# Autodesk Inventor assembly: Build Platform Assembly 1.0
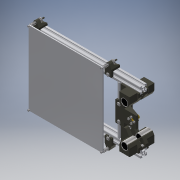
[picture p0: Inventor's stored thumbnail of the model, 180x180]
Saved by Autodesk Inventor 2016 (Build 200138000, 138)
## iProperties
Created: 2017-04-13
Part Number: Build Platform Assembly 1.0
Document SubType Name: Assembly
Designer: Scott
Author: Scott
## Documents named in this file (16)
- E:\Scott Projects\3D Printing\CoreXY\Build Platform Assembly 1.0.iam
- E:\Scott Projects\3D Printing\CoreXY\2020 Extrusion - Bed rear.ipt
- E:\Scott Projects\3D Printing\CoreXY\Z Axis Bearing Holder 1.0.ipt
- E:\Scott Projects\3D Printing\CoreXY\2020 Extrusion - Bed sides.ipt
- E:\Scott Projects\3D Printing\CoreXY\LM12UU.ipt
- E:\Scott Projects\3D Printing\CoreXY\Heated Bed.ipt
- E:\Scott Projects\3D Printing\CoreXY\Mk2 Heat Bed Bracket.ipt
- C:\Users\Scott\Documents\Inventor\Content Center Files\R2016\en-US\ANSI B18.3.4M(1)\ANSI B18.3.4M - M5 x 0.8 x 10(2).ipt
- C:\Users\Scott\Documents\Inventor\Content Center Files\R2016\en-US\ANSI B18.3.1M(1)\ANSI B18.3.1M - M3x0.5 x 40(2).ipt
- E:\Scott Projects\3D Printing\CoreXY\Bed spring.ipt
- E:\Scott Projects\3D Printing\CoreXY\Bed Thumb Screw.ipt
- E:\Scott Projects\3D Printing\CoreXY\Z Nut Braket 1.0.ipt
- E:\Scott Projects\3D Printing\CoreXY\Trapezoidal lead screw Nut tr8x8-4.ipt
- C:\Users\Scott\Documents\Inventor\Content Center Files\R2016\en-US\ANSI B18.3.1M(1)\ANSI B18.3.1M - M3x0.5 x 12(2).ipt
- C:\Users\Scott\Documents\Inventor\Content Center Files\R2016\en-US\ISO 4032(2)\ISO 4032 - M3 - ISO.ipt
- E:\Scott Projects\3D Printing\CoreXY\HyperCube parameters.xlsx
## Components (56 placed, 14 different names)
1. 2020 Extrusion - Bed rear:1 — Flush:1, Flush:2, Flush:3, Mate:1, Flush:4, Mate:2, Mate:3, Mate:4, Flush:5, Mate:10, Mate:28, Mate:29
2. Z Axis Bearing Holder 1.0:1 — Mate:3, Mate:4, Flush:5, Mate:5, Mate:6, Flush:7, Insert:2, Insert:4, Insert:26, Insert:27, Insert:28, Insert:29
3. Z Axis Bearing Holder 1.0:2 — Mate:1, Flush:4, Mate:2, Mate:7, Mate:8, Flush:6, Insert:1, Insert:3, Insert:22, Insert:23, Insert:24, Insert:25
4. 2020 Extrusion - Bed sides:1 — Mate:5, Mate:6, Flush:7, Mate:9, Mate:18, Mate:19, Mate:21, Mate:22
5. 2020 Extrusion - Bed sides:2 — Mate:7, Mate:8, Flush:6, Mate:12, Mate:13, Mate:15, Mate:16
6. LM12UU:1 — Insert:4
7. LM12UU:2 — Insert:3
8. LM12UU:3 — Insert:2
9. LM12UU:4 — Insert:1, Mate:11
10. Heated Bed:1 — Mate:9, Mate:10, Mate:11, Mate:14, Mate:17, Mate:20, Mate:23, Insert:13, Insert:14, Insert:15, Insert:16
11. Mk2 Heat Bed Bracket:1 — Mate:12, Mate:13, Mate:14, Insert:11, Insert:12, Flush:9, Insert:20
12. Mk2 Heat Bed Bracket:2 — Mate:15, Mate:16, Mate:17, Insert:9, Insert:10, Flush:8, Insert:19
13. Mk2 Heat Bed Bracket:3 — Mate:21, Mate:22, Mate:23, Insert:5, Flush:10, Insert:18, Insert:21
14. Mk2 Heat Bed Bracket:4 — Mate:18, Mate:19, Mate:20, Insert:7, Insert:8, Flush:11, Insert:17
15. Broached Hexagon Socket Button Head Cap Screw - Metric M5 x 0.8 x 10:1 — Insert:9
16. Broached Hexagon Socket Button Head Cap Screw - Metric M5 x 0.8 x 10:2 — Insert:12
17. Broached Hexagon Socket Button Head Cap Screw - Metric M5 x 0.8 x 10:3 — Insert:8
18. Broached Hexagon Socket Button Head Cap Screw - Metric M5 x 0.8 x 10:4 — Insert:11
19. Broached Hexagon Socket Button Head Cap Screw - Metric M5 x 0.8 x 10:5 — Insert:7
20. Broached Hexagon Socket Button Head Cap Screw - Metric M5 x 0.8 x 10:6 — Insert:10
21. Broached Hexagon Socket Button Head Cap Screw - Metric M5 x 0.8 x 10:7 — Insert:5
22. Broached Hexagon Socket Button Head Cap Screw - Metric M5 x 0.8 x 10:8 — Insert:21
23. Broached Socket Head Cap Screw - Metric M3x0.5 x 40:1 — Insert:16, Mate:27
24. Broached Socket Head Cap Screw - Metric M3x0.5 x 40:2 — Insert:15, Mate:26
25. Broached Socket Head Cap Screw - Metric M3x0.5 x 40:3 — Insert:14, Mate:25
26. Broached Socket Head Cap Screw - Metric M3x0.5 x 40:4 — Insert:13, Mate:24
27. Bed spring:1 — Mate:24, Flush:8
28. Bed spring:2 — Mate:25, Flush:9
29. Bed spring:3 — Mate:26, Flush:10
30. Bed spring:4 — Mate:27, Flush:11
31. Bed Thumb Screw:1 — Insert:19
32. Bed Thumb Screw:2 — Insert:17
33. Bed Thumb Screw:3 — Insert:20
34. Bed Thumb Screw:4 — Insert:18
35. Broached Hexagon Socket Button Head Cap Screw - Metric M5 x 0.8 x 10:9 — Insert:22
36. Broached Hexagon Socket Button Head Cap Screw - Metric M5 x 0.8 x 10:10 — Insert:23
37. Broached Hexagon Socket Button Head Cap Screw - Metric M5 x 0.8 x 10:11 — Insert:24
38. Broached Hexagon Socket Button Head Cap Screw - Metric M5 x 0.8 x 10:12 — Insert:25
39. Broached Hexagon Socket Button Head Cap Screw - Metric M5 x 0.8 x 10:13 — Insert:29
40. Broached Hexagon Socket Button Head Cap Screw - Metric M5 x 0.8 x 10:14 — Insert:28
41. Broached Hexagon Socket Button Head Cap Screw - Metric M5 x 0.8 x 10:15 — Insert:27
42. Broached Hexagon Socket Button Head Cap Screw - Metric M5 x 0.8 x 10:16 — Insert:26
43. Z Nut Braket 1.0:1 — Mate:28, Mate:29, Flush:12, Insert:30, Insert:31, Insert:32, Insert:33, Mate:31, Mate:34, Mate:35, Mate:37, Mate:39, Angle:1, Angle:2, Angle:3, Angle:4, Mate:41
44. Broached Hexagon Socket Button Head Cap Screw - Metric M5 x 0.8 x 10:17 — Insert:31
45. Broached Hexagon Socket Button Head Cap Screw - Metric M5 x 0.8 x 10:18 — Insert:30
46. Broached Hexagon Socket Button Head Cap Screw - Metric M5 x 0.8 x 10:19 — Insert:32
47. Broached Hexagon Socket Button Head Cap Screw - Metric M5 x 0.8 x 10:20 — Insert:33
48. Trapezoidal lead screw Nut tr8x8-4:1 — Mate:30, Mate:31, Mate:32, Mate:33, Mate:36, Mate:38, Mate:40, Insert:34, Insert:35, Insert:36, Insert:37, Mate:41
49. Broached Socket Head Cap Screw - Metric M3x0.5 x 12:1 — Mate:33, Mate:34
50. Broached Socket Head Cap Screw - Metric M3x0.5 x 12:2 — Mate:39, Mate:40
51. Broached Socket Head Cap Screw - Metric M3x0.5 x 12:3 — Mate:37, Mate:38
52. Broached Socket Head Cap Screw - Metric M3x0.5 x 12:4 — Mate:35, Mate:36
53. ISO 4032 M3:1 — Insert:34, Angle:1
54. ISO 4032 M3:2 — Insert:36, Angle:4
55. ISO 4032 M3:3 — Insert:37, Angle:2
56. ISO 4032 M3:4 — Insert:35, Angle:3
## Relationships (93: Mate 41, Insert 36, Flush 12, Angle 4)
- Flush:1: 2020 Extrusion - Bed rear:1
- Flush:2 (0.2 mm): 2020 Extrusion - Bed rear:1
- Flush:3: 2020 Extrusion - Bed rear:1
- Mate:1: 2020 Extrusion - Bed rear:1 ↔ Z Axis Bearing Holder 1.0:2
- Flush:4: 2020 Extrusion - Bed rear:1 ↔ Z Axis Bearing Holder 1.0:2
- Mate:2 (0.2 mm): 2020 Extrusion - Bed rear:1 ↔ Z Axis Bearing Holder 1.0:2
- Mate:3: 2020 Extrusion - Bed rear:1 ↔ Z Axis Bearing Holder 1.0:1
- Mate:4: 2020 Extrusion - Bed rear:1 ↔ Z Axis Bearing Holder 1.0:1
- Flush:5: 2020 Extrusion - Bed rear:1 ↔ Z Axis Bearing Holder 1.0:1
- Mate:5: Z Axis Bearing Holder 1.0:1 ↔ 2020 Extrusion - Bed sides:1
- Mate:6 (0.2 mm): Z Axis Bearing Holder 1.0:1 ↔ 2020 Extrusion - Bed sides:1
- Mate:7: Z Axis Bearing Holder 1.0:2 ↔ 2020 Extrusion - Bed sides:2
- Mate:8 (0.2 mm): Z Axis Bearing Holder 1.0:2 ↔ 2020 Extrusion - Bed sides:2
- Flush:6: Z Axis Bearing Holder 1.0:2 ↔ 2020 Extrusion - Bed sides:2
- Flush:7: Z Axis Bearing Holder 1.0:1 ↔ 2020 Extrusion - Bed sides:1
- Insert:1: Z Axis Bearing Holder 1.0:2 ↔ LM12UU:4
- Insert:2: Z Axis Bearing Holder 1.0:1 ↔ LM12UU:3
- Insert:3: Z Axis Bearing Holder 1.0:2 ↔ LM12UU:2
- Insert:4: Z Axis Bearing Holder 1.0:1 ↔ LM12UU:1
- Mate:9 (20 mm): 2020 Extrusion - Bed sides:1 ↔ Heated Bed:1
- Mate:10: 2020 Extrusion - Bed rear:1 ↔ Heated Bed:1
- Mate:11 (-173.25 mm): LM12UU:4 ↔ Heated Bed:1
- Mate:12: 2020 Extrusion - Bed sides:2 ↔ Mk2 Heat Bed Bracket:1
- Mate:13: 2020 Extrusion - Bed sides:2 ↔ Mk2 Heat Bed Bracket:1
- Mate:14: Heated Bed:1 ↔ Mk2 Heat Bed Bracket:1
- Mate:15: 2020 Extrusion - Bed sides:2 ↔ Mk2 Heat Bed Bracket:2
- Mate:16: 2020 Extrusion - Bed sides:2 ↔ Mk2 Heat Bed Bracket:2
- Mate:17: Heated Bed:1 ↔ Mk2 Heat Bed Bracket:2
- Mate:18: 2020 Extrusion - Bed sides:1 ↔ Mk2 Heat Bed Bracket:4
- Mate:19: 2020 Extrusion - Bed sides:1 ↔ Mk2 Heat Bed Bracket:4
- Mate:20: Heated Bed:1 ↔ Mk2 Heat Bed Bracket:4
- Mate:21: 2020 Extrusion - Bed sides:1 ↔ Mk2 Heat Bed Bracket:3
- Mate:22: 2020 Extrusion - Bed sides:1 ↔ Mk2 Heat Bed Bracket:3
- Mate:23: Heated Bed:1 ↔ Mk2 Heat Bed Bracket:3
- Insert:5: Mk2 Heat Bed Bracket:3 ↔ Broached Hexagon Socket Button Head Cap Screw - Metric M5 x 0.8 x 10:7
- Insert:7: Mk2 Heat Bed Bracket:4 ↔ Broached Hexagon Socket Button Head Cap Screw - Metric M5 x 0.8 x 10:5
- Insert:8: Mk2 Heat Bed Bracket:4 ↔ Broached Hexagon Socket Button Head Cap Screw - Metric M5 x 0.8 x 10:3
- Insert:9: Mk2 Heat Bed Bracket:2 ↔ Broached Hexagon Socket Button Head Cap Screw - Metric M5 x 0.8 x 10:1
- Insert:10: Mk2 Heat Bed Bracket:2 ↔ Broached Hexagon Socket Button Head Cap Screw - Metric M5 x 0.8 x 10:6
- Insert:11: Mk2 Heat Bed Bracket:1 ↔ Broached Hexagon Socket Button Head Cap Screw - Metric M5 x 0.8 x 10:4
- Insert:12: Mk2 Heat Bed Bracket:1 ↔ Broached Hexagon Socket Button Head Cap Screw - Metric M5 x 0.8 x 10:2
- Insert:13: Heated Bed:1 ↔ Broached Socket Head Cap Screw - Metric M3x0.5 x 40:4
- Insert:14: Heated Bed:1 ↔ Broached Socket Head Cap Screw - Metric M3x0.5 x 40:3
- Insert:15: Heated Bed:1 ↔ Broached Socket Head Cap Screw - Metric M3x0.5 x 40:2
- Insert:16: Heated Bed:1 ↔ Broached Socket Head Cap Screw - Metric M3x0.5 x 40:1
- Mate:24: Broached Socket Head Cap Screw - Metric M3x0.5 x 40:4 ↔ Bed spring:1
- Flush:8: Mk2 Heat Bed Bracket:2 ↔ Bed spring:1
- Mate:25: Broached Socket Head Cap Screw - Metric M3x0.5 x 40:3 ↔ Bed spring:2
- Flush:9: Mk2 Heat Bed Bracket:1 ↔ Bed spring:2
- Mate:26: Broached Socket Head Cap Screw - Metric M3x0.5 x 40:2 ↔ Bed spring:3
- Flush:10: Mk2 Heat Bed Bracket:3 ↔ Bed spring:3
- Mate:27: Broached Socket Head Cap Screw - Metric M3x0.5 x 40:1 ↔ Bed spring:4
- Flush:11: Mk2 Heat Bed Bracket:4 ↔ Bed spring:4
- Insert:17: Mk2 Heat Bed Bracket:4 ↔ Bed Thumb Screw:2
- Insert:18: Mk2 Heat Bed Bracket:3 ↔ Bed Thumb Screw:4
- Insert:19: Mk2 Heat Bed Bracket:2 ↔ Bed Thumb Screw:1
- Insert:20: Mk2 Heat Bed Bracket:1 ↔ Bed Thumb Screw:3
- Insert:21: Mk2 Heat Bed Bracket:3 ↔ Broached Hexagon Socket Button Head Cap Screw - Metric M5 x 0.8 x 10:8
- Insert:22: Z Axis Bearing Holder 1.0:2 ↔ Broached Hexagon Socket Button Head Cap Screw - Metric M5 x 0.8 x 10:9
- Insert:23: Z Axis Bearing Holder 1.0:2 ↔ Broached Hexagon Socket Button Head Cap Screw - Metric M5 x 0.8 x 10:10
- Insert:24: Z Axis Bearing Holder 1.0:2 ↔ Broached Hexagon Socket Button Head Cap Screw - Metric M5 x 0.8 x 10:11
- Insert:25: Z Axis Bearing Holder 1.0:2 ↔ Broached Hexagon Socket Button Head Cap Screw - Metric M5 x 0.8 x 10:12
- Insert:26: Z Axis Bearing Holder 1.0:1 ↔ Broached Hexagon Socket Button Head Cap Screw - Metric M5 x 0.8 x 10:16
- Insert:27: Z Axis Bearing Holder 1.0:1 ↔ Broached Hexagon Socket Button Head Cap Screw - Metric M5 x 0.8 x 10:15
- Insert:28: Z Axis Bearing Holder 1.0:1 ↔ Broached Hexagon Socket Button Head Cap Screw - Metric M5 x 0.8 x 10:14
- Insert:29: Z Axis Bearing Holder 1.0:1 ↔ Broached Hexagon Socket Button Head Cap Screw - Metric M5 x 0.8 x 10:13
- Mate:28: 2020 Extrusion - Bed rear:1 ↔ Z Nut Braket 1.0:1
- Mate:29: 2020 Extrusion - Bed rear:1 ↔ Z Nut Braket 1.0:1
- Flush:12: Z Nut Braket 1.0:1
- Insert:30: Z Nut Braket 1.0:1 ↔ Broached Hexagon Socket Button Head Cap Screw - Metric M5 x 0.8 x 10:18
- Insert:31: Z Nut Braket 1.0:1 ↔ Broached Hexagon Socket Button Head Cap Screw - Metric M5 x 0.8 x 10:17
- Insert:32: Z Nut Braket 1.0:1 ↔ Broached Hexagon Socket Button Head Cap Screw - Metric M5 x 0.8 x 10:19
- Insert:33: Z Nut Braket 1.0:1 ↔ Broached Hexagon Socket Button Head Cap Screw - Metric M5 x 0.8 x 10:20
- Mate:30: Trapezoidal lead screw Nut tr8x8-4:1
- Mate:31: Z Nut Braket 1.0:1 ↔ Trapezoidal lead screw Nut tr8x8-4:1
- Mate:32: Trapezoidal lead screw Nut tr8x8-4:1
- Mate:33: Trapezoidal lead screw Nut tr8x8-4:1 ↔ Broached Socket Head Cap Screw - Metric M3x0.5 x 12:1
- Mate:34: Z Nut Braket 1.0:1 ↔ Broached Socket Head Cap Screw - Metric M3x0.5 x 12:1
- Mate:35: Z Nut Braket 1.0:1 ↔ Broached Socket Head Cap Screw - Metric M3x0.5 x 12:4
- Mate:36: Trapezoidal lead screw Nut tr8x8-4:1 ↔ Broached Socket Head Cap Screw - Metric M3x0.5 x 12:4
- Mate:37: Z Nut Braket 1.0:1 ↔ Broached Socket Head Cap Screw - Metric M3x0.5 x 12:3
- Mate:38: Trapezoidal lead screw Nut tr8x8-4:1 ↔ Broached Socket Head Cap Screw - Metric M3x0.5 x 12:3
- Mate:39: Z Nut Braket 1.0:1 ↔ Broached Socket Head Cap Screw - Metric M3x0.5 x 12:2
- Mate:40: Trapezoidal lead screw Nut tr8x8-4:1 ↔ Broached Socket Head Cap Screw - Metric M3x0.5 x 12:2
- Insert:34: Trapezoidal lead screw Nut tr8x8-4:1 ↔ ISO 4032 M3:1
- Insert:35: Trapezoidal lead screw Nut tr8x8-4:1 ↔ ISO 4032 M3:4
- Insert:36: Trapezoidal lead screw Nut tr8x8-4:1 ↔ ISO 4032 M3:2
- Insert:37: Trapezoidal lead screw Nut tr8x8-4:1 ↔ ISO 4032 M3:3
- Angle:1 (0 deg): Z Nut Braket 1.0:1 ↔ ISO 4032 M3:1
- Angle:2 (0 deg): Z Nut Braket 1.0:1 ↔ ISO 4032 M3:3
- Angle:3 (0 deg): Z Nut Braket 1.0:1 ↔ ISO 4032 M3:4
- Angle:4 (0 deg): Z Nut Braket 1.0:1 ↔ ISO 4032 M3:2
- Mate:41 (-14 mm): Z Nut Braket 1.0:1 ↔ Trapezoidal lead screw Nut tr8x8-4:1
## Named parameters: extrusion_size = 30 mm, frame_width = 400 mm, frame_depth = 380 mm, frame_height = 400 mm, platform_width = 214 mm, platform_depth = 214 mm, hole_spacing_width = 210 mm, hole_spacing_depth = 210 mm, bed_extrusion_size = 20 mm, bed_frame_width = 180 mm, bed_frame_depth = 310 mm, bed_cl_y_offset = 173.25 mm, T8_screw_length = 250 mm
